# Autodesk Inventor assembly: ToolLockAssy
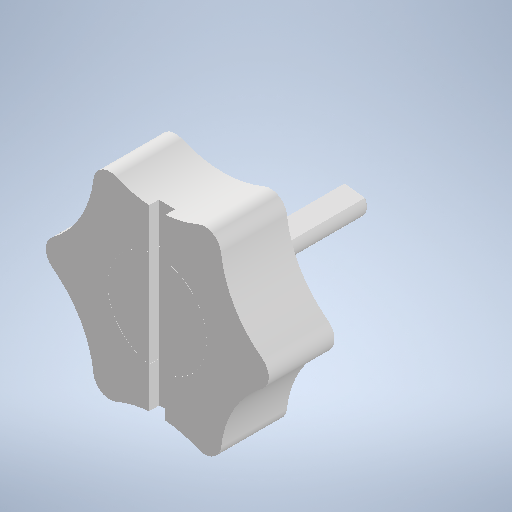
[picture p0: Inventor's stored thumbnail of the model, 512x512]
Saved by Autodesk Inventor 2025.3 (Build 293356030, 356C)
## iProperties
Created: 2025-10-10
Part Number: ToolLockAssy
Document SubType Name: Assembly
Designer: tvoko
Author: tvoko
## Documents named in this file (4)
- C:\Users\tvoko\Github\DIY-Coil-Winder\CAD\ToolLockAssy.iam
- C:\Users\tvoko\Github\DIY-Coil-Winder\CAD\Tool-lock-Slot.ipt
- C:\Users\tvoko\Github\DIY-Coil-Winder\CAD\Tool-Lock-Knob.ipt
- C:\Users\tvoko\Github\DIY-Coil-Winder\CAD\8mm D-Shaft axle (3d print).ipt
## Components (3 placed, 3 different names)
1. Tool-lock-Slot:1 — Mate:1, Mate:2, Mate:3, Mate:5, Mate:6, Mate:7
2. Tool-Lock-Knob:1 — Mate:1, Mate:2, Mate:3, Mate:4, Tangent:1, Tangent:2, Tangent:3, Mate:7
3. 8mm D-Shaft axle (3d print):1 — Mate:5, Mate:6
## Relationships (10: Mate 7, Tangent 3)
- Mate:1: Tool-lock-Slot:1 ↔ Tool-Lock-Knob:1
- Mate:2: Tool-lock-Slot:1 ↔ Tool-Lock-Knob:1
- Mate:3: Tool-lock-Slot:1 ↔ Tool-Lock-Knob:1
- Mate:4: Tool-Lock-Knob:1
- Tangent:1: Tool-Lock-Knob:1
- Tangent:2: Tool-Lock-Knob:1
- Tangent:3: Tool-Lock-Knob:1
- Mate:5: Tool-lock-Slot:1 ↔ 8mm D-Shaft axle (3d print):1
- Mate:6: Tool-lock-Slot:1 ↔ 8mm D-Shaft axle (3d print):1
- Mate:7: Tool-lock-Slot:1 ↔ Tool-Lock-Knob:1
